# Autodesk Inventor assembly: Frame
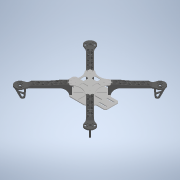
[picture p0: Inventor's stored thumbnail of the model, 180x180]
Saved by Autodesk Inventor 2020 (Build 240168000, 168)
## iProperties
Created: 2019-06-13
Part Number: Frame
Document SubType Name: Assembly
Designer: amirt
Author: amirt
## Documents named in this file (4)
- C:\Users\amirt\Documents\Inventor\Drone\Frame.iam
- C:\Users\amirt\Documents\Inventor\Drone\F330 low plate v1.ipt
- C:\Users\amirt\Documents\Inventor\Drone\DJI F330 qoadrotor arm.iam
- C:\Users\amirt\Documents\Inventor\Drone\F330 Top plate2 v1.ipt
## Components (6 placed, 3 different names)
1. F330 low plate v1:1 — Tangent:3, Tangent:4, Mate:1
2. F330 Top plate2 v1:1 — Insert:1, Mate:2
3. DJI F330 qoadrotor arm:1 [sub-assembly] — Tangent:3, Tangent:4, Mate:1
4. DJI F330 qoadrotor arm:2 [sub-assembly]
5. DJI F330 qoadrotor arm:3 [sub-assembly]
6. DJI F330 qoadrotor arm:4 [sub-assembly] — Insert:1, Mate:2
## Component patterns: (4 elements, first: DJI F330 qoadrotor arm:1)
## Relationships (5: Tangent 2, Mate 2, Insert 1)
- Tangent:3: F330 low plate v1:1 ↔ DJI F330 qoadrotor arm:1
- Tangent:4: F330 low plate v1:1 ↔ DJI F330 qoadrotor arm:1
- Mate:1: F330 low plate v1:1 ↔ DJI F330 qoadrotor arm:1
- Insert:1: F330 Top plate2 v1:1 ↔ DJI F330 qoadrotor arm:4
- Mate:2: F330 Top plate2 v1:1 ↔ DJI F330 qoadrotor arm:4
